# Autodesk Inventor assembly: flip down asmb
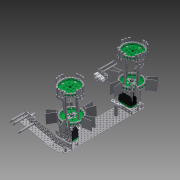
[picture p0: Inventor's stored thumbnail of the model, 180x180]
Saved by Autodesk Inventor 2014 SP1 (Build 180222100, 222)
## iProperties
Created: 2014-04-03
Part Number: flip down asmb
Document SubType Name: Assembly
Designer: Ryan
Author: Ryan
## Documents named in this file (8)
- C:\Users\Ryan\Desktop\sw\toss up 5th A bot\intake\flip down asmb.iam
- C:\Users\Ryan\Desktop\sw\lib\Aperture VEX CAD Library\Metal\Plate\5 x 25.ipt
- C:\Users\Ryan\Desktop\sw\toss up 5th A bot\intake\one roller asmb.iam
- C:\Users\Ryan\Desktop\sw\toss up 5th A bot\intake\plate attachment .iam
- C:\Users\Ryan\Desktop\sw\toss up 5th A bot\intake\spinning thing.iam
- C:\Users\Ryan\Desktop\sw\toss up 5th A bot\intake\one roller asmb_MIR.iam
- C:\Users\Ryan\Desktop\sw\toss up 5th A bot\intake\rubber band holder.iam
- C:\Users\Ryan\Desktop\sw\toss up 5th A bot\intake\plate attachment _MIR.iam
## Components (9 placed, 7 different names)
1. 5 x 25:1 — Mate:1, Mate:2, Mate:3, Mate:4, Mate:5, Mate:6, Flush:1, Flush:2, Flush:3, Mate:11, Mate:12, Mate:13, Mate:14, Mate:15, Mate:16, Angle:1, Angle:2
2. one roller asmb:1 [sub-assembly] — Mate:1, Mate:2, Mate:3, Mate:4, Mate:5, Mate:7, Mate:8
3. plate attachment :1 [sub-assembly] — Mate:6, Flush:1, Flush:2
4. spinning thing:1 [sub-assembly] — Mate:7, Mate:8
5. one roller asmb_MIR:1 [sub-assembly] — Mate:9, Mate:10
6. spinning thing:2 [sub-assembly] — Mate:9, Mate:10
7. rubber band holder:1 [sub-assembly] — Mate:11, Mate:12, Mate:13, Angle:2
8. rubber band holder:2 [sub-assembly] — Mate:14, Mate:15, Mate:16, Angle:1
9. plate attachment _MIR:1 [sub-assembly]
## Relationships (21: Mate 16, Flush 3, Angle 2)
- Mate:1: 5 x 25:1 ↔ one roller asmb:1
- Mate:2 (2.3114 mm): 5 x 25:1 ↔ one roller asmb:1
- Mate:3 (2.3114 mm): 5 x 25:1 ↔ one roller asmb:1
- Mate:4 (2.3114 mm): 5 x 25:1 ↔ one roller asmb:1
- Mate:5 (2.3114 mm): 5 x 25:1 ↔ one roller asmb:1
- Mate:6: 5 x 25:1 ↔ plate attachment :1
- Flush:1: 5 x 25:1 ↔ plate attachment :1
- Flush:2: 5 x 25:1 ↔ plate attachment :1
- Mate:7: one roller asmb:1 ↔ spinning thing:1
- Mate:8: one roller asmb:1 ↔ spinning thing:1
- Flush:3 (-158.75 mm): 5 x 25:1
- Mate:9: one roller asmb_MIR:1 ↔ spinning thing:2
- Mate:10: one roller asmb_MIR:1 ↔ spinning thing:2
- Mate:11: 5 x 25:1 ↔ rubber band holder:1
- Mate:12 (2.3114 mm): 5 x 25:1 ↔ rubber band holder:1
- Mate:13 (2.3114 mm): 5 x 25:1 ↔ rubber band holder:1
- Mate:14 (2.3114 mm): 5 x 25:1 ↔ rubber band holder:2
- Mate:15 (2.3114 mm): 5 x 25:1 ↔ rubber band holder:2
- Mate:16: 5 x 25:1 ↔ rubber band holder:2
- Angle:1 (0 deg): 5 x 25:1 ↔ rubber band holder:2
- Angle:2 (0 deg): 5 x 25:1 ↔ rubber band holder:1
## Named parameters: q = 2.3114 mm
